# Autodesk Inventor assembly: Ensamble tablero
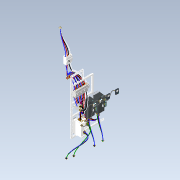
[picture p0: Inventor's stored thumbnail of the model, 180x180]
Saved by Autodesk Inventor 2021 (Build 250183000, 183)
## iProperties
Created: 2021-08-22
Part Number: Ensamble tablero
Document SubType Name: Assembly
Designer: Andrés Holguín
Author: Andrés Holguín
## Documents named in this file (32)
- C:\Users\andre\Documents\GitHub\Dis.-Mecatronico-E6\inventor proyecto\Tablero\Ensamble tablero.iam
- C:\Users\andre\Documents\GitHub\Dis.-Mecatronico-E6\inventor proyecto\Tablero\Interruptores\3p30.ipt
- C:\Users\andre\Documents\GitHub\Dis.-Mecatronico-E6\inventor proyecto\Tablero\Interruptores\3p50.ipt
- C:\Users\andre\Documents\GitHub\Dis.-Mecatronico-E6\inventor proyecto\Tablero\Interruptores\2p8\a9n18344.iam
- C:\Users\andre\Documents\GitHub\Dis.-Mecatronico-E6\inventor proyecto\Tablero\Riel DIN\Riel DIN.ipt
- C:\Users\andre\Documents\GitHub\Dis.-Mecatronico-E6\inventor proyecto\Tablero\Variador\G120_G120_3D_3654a134dd9c4e348126222df3348349.iam
- C:\Users\andre\Documents\GitHub\Dis.-Mecatronico-E6\inventor proyecto\Tablero\DriveAvance\PARTserver0202108230417182353949810e898ce\AIS2021\5340825 CMMT-AS-C4-3A-EP-S1.iam
- C:\Users\andre\Documents\GitHub\Dis.-Mecatronico-E6\inventor proyecto\Tablero\DriveActuador\AIS2021\8133356 CMMT-AS-C7-11A-P3-EP-S1.iam
- C:\Users\andre\Documents\GitHub\Dis.-Mecatronico-E6\inventor proyecto\Tablero\DriveActuador\2247681 CACN-3A-1-5.ipt
- C:\Users\andre\Documents\GitHub\Dis.-Mecatronico-E6\inventor proyecto\Tablero\Interruptores\2p15.ipt
- C:\Users\andre\Documents\GitHub\Dis.-Mecatronico-E6\inventor proyecto\Tablero\Extra\pin.ipt
- C:\Users\andre\Documents\GitHub\Dis.-Mecatronico-E6\inventor proyecto\Tablero\Variador\IOP-2_SINAMICS_G_V_6SL3255-0AA00-4JA2_3D_836dc0bd695c2b03fe1a6a7dff666d83.ipt
- C:\Users\andre\Documents\GitHub\Dis.-Mecatronico-E6\inventor proyecto\Tablero\AIS2021\5065802 6GD-1RR7_62-CLP-CBL.ipt
- C:\Users\andre\Documents\GitHub\Dis.-Mecatronico-E6\inventor proyecto\Tablero\AIS2021\5065608 2GD-1RR5,08-CLP-CBL.ipt
- C:\Users\andre\Documents\GitHub\Dis.-Mecatronico-E6\inventor proyecto\Tablero\AIS2021\5065752 4GD-1RR7_62-CLP-CBL.ipt
- C:\Users\andre\Documents\GitHub\Dis.-Mecatronico-E6\inventor proyecto\Tablero\AIS2021\3943133 4GD-1RR5,08-CLP-CBL.ipt
- C:\Users\andre\Documents\GitHub\Dis.-Mecatronico-E6\inventor proyecto\Tablero\AIS2021\4280684 14RD-1RR5_08-CLP-CBL.ipt
- C:\Users\andre\Documents\GitHub\Dis.-Mecatronico-E6\inventor proyecto\Tablero\Ensamble tablero.Harness1.iam
- C:\Users\andre\Documents\GitHub\Dis.-Mecatronico-E6\inventor proyecto\Tablero\DriveActuador\8070984 CDSB-A1.ipt
- C:\Users\andre\Documents\GitHub\Dis.-Mecatronico-E6\inventor proyecto\Tablero\Interruptores\4p180.ipt
- C:\Users\andre\Documents\GitHub\Dis.-Mecatronico-E6\inventor proyecto\Tablero\Riel DIN\Riel DIN 2.ipt
- C:\Users\andre\Documents\GitHub\Dis.-Mecatronico-E6\inventor proyecto\Tablero\Canaletas\canaletaIzquierda.iam
- C:\Users\andre\Documents\GitHub\Dis.-Mecatronico-E6\inventor proyecto\Tablero\Canaletas\canaletaInferior.iam
- C:\Users\andre\Documents\GitHub\Dis.-Mecatronico-E6\inventor proyecto\Tablero\Canaletas\canaletaDerecha.iam
- C:\Users\andre\Documents\GitHub\Dis.-Mecatronico-E6\inventor proyecto\Tablero\Canaletas\canaletaSuperior.iam
- C:\Users\andre\Documents\GitHub\Dis.-Mecatronico-E6\inventor proyecto\Tablero\Canaletas\canaletaMedia.iam
- C:\Users\andre\Documents\GitHub\Dis.-Mecatronico-E6\inventor proyecto\Tablero\Canaletas\canaletaVar.iam
- C:\Users\andre\Documents\GitHub\Dis.-Mecatronico-E6\inventor proyecto\Tablero\Bloque distribucion\lgy416048.iam
- C:\Users\andre\Documents\GitHub\Dis.-Mecatronico-E6\inventor proyecto\Tablero\Canaletas\canaletaInt.iam
- C:\Users\andre\Documents\GitHub\Dis.-Mecatronico-E6\inventor proyecto\Tablero\Canaletas\canaletaMenor.iam
- C:\Users\andre\Documents\GitHub\Dis.-Mecatronico-E6\inventor proyecto\Tablero\Canaletas\canaleta2.iam
- C:\Users\andre\Documents\GitHub\Dis.-Mecatronico-E6\inventor proyecto\Tablero\Canaletas\canaleta3.iam
## Components (40 placed, 31 different names)
1. 3p30:1 — Rigid:2, Rigid:3
2. 3p50:2 — Rigid:1, Mate:1, Rigid:2
3. 3p50:1 — Rigid:1
4. a9n18344:1 [sub-assembly] — Rigid:4
5. Riel DIN:1 — Mate:1
6. G120_G120_3D_3654a134dd9c4e348126222df3348349:1 [sub-assembly]
7. G120_G120_3D_3654a134dd9c4e348126222df3348349:2 [sub-assembly]
8. 5340825 CMMT-AS-C4-3A-EP-S1:1 [sub-assembly] — Rigid:9, Rigid:11
9. 8133356 CMMT-AS-C7-11A-P3-EP-S1:1 [sub-assembly] — Rigid:6, Rigid:7, Rigid:10
10. 2247681 CACN-3A-1-5:1 — Mate:2
11. 2p15:1 — Rigid:3, Rigid:4
12. pin:1
13. pin:2
14. pin:3
15. IOP-2_SINAMICS_G_V_6SL3255-0AA00-4JA2_3D_836dc0bd695c2b03fe1a6a7dff666d83:1
16. IOP-2_SINAMICS_G_V_6SL3255-0AA00-4JA2_3D_836dc0bd695c2b03fe1a6a7dff666d83:2
17. 5065802 6GD-1RR7_62-CLP-CBL:1 — Rigid:6
18. 5065608 2GD-1RR5,08-CLP-CBL:1 — Rigid:10
19. 5065752 4GD-1RR7_62-CLP-CBL:1 — Rigid:7
20. 3943133 4GD-1RR5,08-CLP-CBL:1 — Rigid:11
21. 4280684 14RD-1RR5_08-CLP-CBL:1 — Rigid:9
22. Harness1 [sub-assembly]
23. 8070984 CDSB-A1:1
24. 8070984 CDSB-A1:2
25. 4p180:1
26. pin:4
27. pin:5
28. Riel DIN 2:1 — Mate:2
29. canaletaIzquierda:1 [sub-assembly] — Rigid:18, Mate:4, Flush:1, Flush:3, Flush:4, Mate:9, Rigid:20, Rigid:21
30. canaletaInferior:1 [sub-assembly] — Rigid:16, Rigid:17, Mate:7, Flush:3, Rigid:20
31. canaletaDerecha:1 [sub-assembly] — Flush:2, Mate:6, Mate:7, Mate:10
32. canaletaSuperior:1 [sub-assembly] — Rigid:18, Rigid:19
33. canaletaMedia:1 [sub-assembly] — Flush:2, Mate:6, Rigid:21
34. canaletaVar:1 [sub-assembly] — Rigid:16
35. canaletaVar:2 [sub-assembly] — Rigid:17
36. lgy416048:1 [sub-assembly]
37. canaletaInt:1 [sub-assembly] — Mate:4, Flush:1, Mate:8, Rigid:22
38. canaletaMenor:1 [sub-assembly] — Rigid:19, Mate:8
39. canaleta2:1 [sub-assembly] — Flush:4, Mate:9, Mate:10
40. canaleta3:1 [sub-assembly] — Rigid:22
## Relationships (28: WeldJoint 16, Mate 8, Flush 4)
- Rigid:1 [WeldJoint]: 3p50:2 ↔ 3p50:1
- Mate:1: 3p50:2 ↔ Riel DIN:1
- Rigid:2 [WeldJoint]: 3p30:1 ↔ 3p50:2
- Rigid:3 [WeldJoint]: 3p30:1 ↔ 2p15:1
- Rigid:4 [WeldJoint]: a9n18344:1 ↔ 2p15:1
- Rigid:6 [WeldJoint]: 8133356 CMMT-AS-C7-11A-P3-EP-S1:1 ↔ 5065802 6GD-1RR7_62-CLP-CBL:1
- Rigid:7 [WeldJoint]: 8133356 CMMT-AS-C7-11A-P3-EP-S1:1 ↔ 5065752 4GD-1RR7_62-CLP-CBL:1
- Rigid:9 [WeldJoint] (2 mm): 5340825 CMMT-AS-C4-3A-EP-S1:1 ↔ 4280684 14RD-1RR5_08-CLP-CBL:1
- Rigid:10 [WeldJoint]: 8133356 CMMT-AS-C7-11A-P3-EP-S1:1 ↔ 5065608 2GD-1RR5,08-CLP-CBL:1
- Rigid:11 [WeldJoint] (1 mm): 5340825 CMMT-AS-C4-3A-EP-S1:1 ↔ 3943133 4GD-1RR5,08-CLP-CBL:1
- Mate:2: 2247681 CACN-3A-1-5:1 ↔ Riel DIN 2:1
- Rigid:16 [WeldJoint]: canaletaInferior:1 ↔ canaletaVar:1
- Rigid:17 [WeldJoint]: canaletaInferior:1 ↔ canaletaVar:2
- Rigid:18 [WeldJoint]: canaletaIzquierda:1 ↔ canaletaSuperior:1
- Rigid:19 [WeldJoint]: canaletaSuperior:1 ↔ canaletaMenor:1
- Mate:4: canaletaIzquierda:1 ↔ canaletaInt:1
- Flush:1: canaletaIzquierda:1 ↔ canaletaInt:1
- Flush:2: canaletaDerecha:1 ↔ canaletaMedia:1
- Mate:6: canaletaDerecha:1 ↔ canaletaMedia:1
- Mate:7: canaletaInferior:1 ↔ canaletaDerecha:1
- Flush:3: canaletaIzquierda:1 ↔ canaletaInferior:1
- Mate:8: canaletaInt:1 ↔ canaletaMenor:1
- Flush:4: canaletaIzquierda:1 ↔ canaleta2:1
- Mate:9: canaletaIzquierda:1 ↔ canaleta2:1
- Mate:10: canaletaDerecha:1 ↔ canaleta2:1
- Rigid:20 [WeldJoint]: canaletaIzquierda:1 ↔ canaletaInferior:1
- Rigid:21 [WeldJoint]: canaletaIzquierda:1 ↔ canaletaMedia:1
- Rigid:22 [WeldJoint]: canaletaInt:1 ↔ canaleta3:1
